# Autodesk Inventor assembly: Full Carousel Assembly
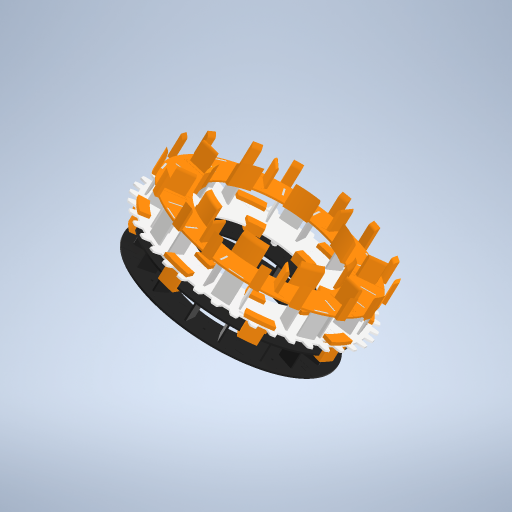
[picture p0: Inventor's stored thumbnail of the model, 512x512]
Saved by Autodesk Inventor 2023 (Build 270158000, 158)
## iProperties
Created: 2023-02-14
Part Number: Full Carousel Assembly
Document SubType Name: Assembly
Designer: cheng
Author: cheng
## Documents named in this file (3)
- C:\Users\cheng\Desktop\4th Year Project\Inventor\12th Assembly\Full Carousel Assembly.iam
- C:\Users\cheng\Desktop\4th Year Project\Inventor\12th Assembly\Moving Carousel\Moving Carousel Assembly.iam
- C:\Users\cheng\Desktop\4th Year Project\Inventor\12th Assembly\Carousel Base Plate Laser Cut\base Plate Laser Full Carou ASSEMBLY.iam
## Components (2 placed, 2 different names)
1. base Plate Laser Full Carou ASSEMBLY:1 [sub-assembly] — Mate:1, Mate:2
2. Moving Carousel Assembly:2 [sub-assembly] — Mate:1, Mate:2
## Relationships (2: Mate 2)
- Mate:1: base Plate Laser Full Carou ASSEMBLY:1 ↔ Moving Carousel Assembly:2
- Mate:2: base Plate Laser Full Carou ASSEMBLY:1 ↔ Moving Carousel Assembly:2
